# Autodesk Inventor assembly: Gantry1
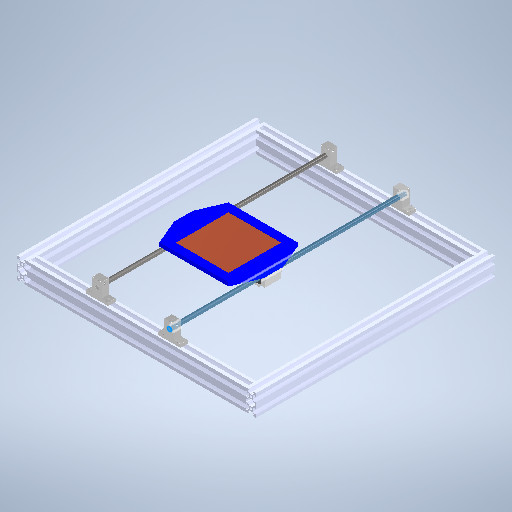
[picture p0: Inventor's stored thumbnail of the model, 512x512]
Saved by Autodesk Inventor 2025.2 (Build 292293000, 293)
## iProperties
Created: 2025-05-31
Part Number: Gantry1
Document SubType Name: Assembly
Designer: Simon
Author: Simon
## Documents named in this file (9)
- C:\Users\Simon\Projects\Hydrogel-3D-Printer\Hardware\Bioprinter Machine Design\Gantry Concept 1\Gantry1.iam
- C:\Users\Simon\Projects\Hydrogel-3D-Printer\Hardware\Bioprinter Machine Design\Gantry Concept 1\SteelShaft_450mm.ipt
- C:\Users\Simon\Projects\Hydrogel-3D-Printer\Hardware\Bioprinter Machine Design\PartsFolder\SK8_LinearShaftSupport.ipt
- C:\Users\Simon\Projects\Hydrogel-3D-Printer\Hardware\Bioprinter Machine Design\PartsFolder\PeltierTEC1_12706.ipt
- C:\Users\Simon\Projects\Hydrogel-3D-Printer\Hardware\Bioprinter Machine Design\PartsFolder\SC8UU\SC8UU.iam
- C:\Users\Simon\Projects\Hydrogel-3D-Printer\Hardware\Bioprinter Machine Design\Gantry Concept 1\BedPlate.ipt
- C:\Users\Simon\Projects\Hydrogel-3D-Printer\Hardware\Bioprinter Machine Design\Gantry Concept 1\BedHousingFrame.ipt
- C:\Users\Simon\Projects\Hydrogel-3D-Printer\Hardware\Bioprinter Machine Design\Gantry Concept 1\2040_AluminimProfile_450.ipt
- C:\Users\Simon\Projects\Hydrogel-3D-Printer\Hardware\Bioprinter Machine Design\Gantry Concept 1\2040_AluminimProfile_410.ipt
## Components (15 placed, 8 different names)
1. SteelShaft_450mm:1 — Mate:1, Mate:3, Flush:1, Flush:4, Mate:5
2. SteelShaft_450mm:2 — Mate:2, Mate:4, Flush:2, Flush:3, Mate:6
3. SK8_LinearShaftSupport:1 — Mate:1, Flush:1, Flush:5, Flush:6, Mate:26
4. SK8_LinearShaftSupport:2 — Mate:2, Flush:2, Flush:5, Flush:6, Mate:23, Flush:19
5. SK8_LinearShaftSupport:3 — Mate:3, Flush:4, Mate:25
6. SK8_LinearShaftSupport:4 — Mate:4, Flush:3, Mate:24
7. PeltierTEC1_12706:1 — Mate:7, Flush:7, Flush:8
8. SC8UU:1 [sub-assembly] — Mate:5, Mate:11, Flush:9, Flush:11, Flush:12
9. SC8UU:2 [sub-assembly] — Mate:6, Flush:10, Mate:12, Flush:11
10. BedPlate:1 — Mate:7, Flush:7, Flush:8, Mate:8, Mate:9, Mate:10
11. BedHousingFrame:1 — Mate:8, Mate:9, Mate:10, Mate:11, Flush:9, Flush:10, Mate:12, Flush:12
12. 2040_AluminimProfile_450:1 — Mate:17, Flush:13, Flush:14, Mate:19, Flush:17, Flush:18, Mate:21
13. 2040_AluminimProfile_450:2 — Mate:18, Flush:15, Flush:16, Mate:23, Mate:24
14. 2040_AluminimProfile_410:1 — Mate:17, Flush:13, Flush:14, Mate:18, Flush:15, Flush:16, Mate:20, Mate:26, Flush:19
15. 2040_AluminimProfile_410:2 — Mate:19, Flush:17, Flush:18, Mate:22, Mate:25
## Relationships (41: Mate 22, Flush 19)
- Mate:1: SteelShaft_450mm:1 ↔ SK8_LinearShaftSupport:1
- Mate:2: SteelShaft_450mm:2 ↔ SK8_LinearShaftSupport:2
- Mate:3: SteelShaft_450mm:1 ↔ SK8_LinearShaftSupport:3
- Mate:4: SteelShaft_450mm:2 ↔ SK8_LinearShaftSupport:4
- Flush:1: SteelShaft_450mm:1 ↔ SK8_LinearShaftSupport:1
- Flush:2: SteelShaft_450mm:2 ↔ SK8_LinearShaftSupport:2
- Flush:3: SteelShaft_450mm:2 ↔ SK8_LinearShaftSupport:4
- Flush:4: SteelShaft_450mm:1 ↔ SK8_LinearShaftSupport:3
- Flush:5: SK8_LinearShaftSupport:1 ↔ SK8_LinearShaftSupport:2
- Flush:6: SK8_LinearShaftSupport:1 ↔ SK8_LinearShaftSupport:2
- Mate:5: SteelShaft_450mm:1 ↔ SC8UU:1
- Mate:6: SteelShaft_450mm:2 ↔ SC8UU:2
- Mate:7: PeltierTEC1_12706:1 ↔ BedPlate:1
- Flush:7 (-30 mm): PeltierTEC1_12706:1 ↔ BedPlate:1
- Flush:8 (30 mm): PeltierTEC1_12706:1 ↔ BedPlate:1
- Mate:8: BedPlate:1 ↔ BedHousingFrame:1
- Mate:9: BedPlate:1 ↔ BedHousingFrame:1
- Mate:10: BedPlate:1 ↔ BedHousingFrame:1
- Mate:11: SC8UU:1 ↔ BedHousingFrame:1
- Flush:9: SC8UU:1 ↔ BedHousingFrame:1
- Flush:10: SC8UU:2 ↔ BedHousingFrame:1
- Mate:12: SC8UU:2 ↔ BedHousingFrame:1
- Flush:11: SC8UU:1 ↔ SC8UU:2
- Flush:12 (50 mm): SC8UU:1 ↔ BedHousingFrame:1
- Mate:17: 2040_AluminimProfile_450:1 ↔ 2040_AluminimProfile_410:1
- Flush:13: 2040_AluminimProfile_450:1 ↔ 2040_AluminimProfile_410:1
- Flush:14: 2040_AluminimProfile_450:1 ↔ 2040_AluminimProfile_410:1
- Mate:18: 2040_AluminimProfile_450:2 ↔ 2040_AluminimProfile_410:1
- Flush:15: 2040_AluminimProfile_450:2 ↔ 2040_AluminimProfile_410:1
- Flush:16: 2040_AluminimProfile_450:2 ↔ 2040_AluminimProfile_410:1
- Mate:19: 2040_AluminimProfile_450:1 ↔ 2040_AluminimProfile_410:2
- Flush:17: 2040_AluminimProfile_450:1 ↔ 2040_AluminimProfile_410:2
- Flush:18: 2040_AluminimProfile_450:1 ↔ 2040_AluminimProfile_410:2
- Mate:20: 2040_AluminimProfile_410:1
- Mate:21: 2040_AluminimProfile_450:1
- Mate:22: 2040_AluminimProfile_410:2
- Mate:23: SK8_LinearShaftSupport:2 ↔ 2040_AluminimProfile_450:2
- Mate:24: SK8_LinearShaftSupport:4 ↔ 2040_AluminimProfile_450:2
- Mate:25: SK8_LinearShaftSupport:3 ↔ 2040_AluminimProfile_410:2
- Mate:26: SK8_LinearShaftSupport:1 ↔ 2040_AluminimProfile_410:1
- Flush:19 (3 mm): SK8_LinearShaftSupport:2 ↔ 2040_AluminimProfile_410:1
